# Autodesk Inventor assembly: Light Saber Inventor Native
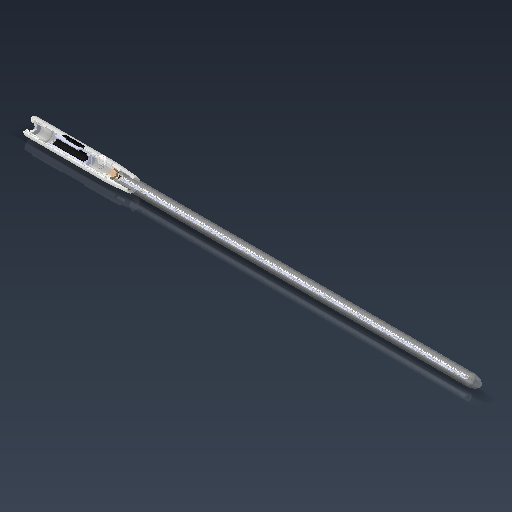
[picture p0: Inventor's stored thumbnail of the model, 512x512]
Saved by Autodesk Inventor 2025.1 (Build 291241000, 241)
## iProperties
Manager: Michael A. Lacey
Company: Personal
Created: 2024-08-20
Part Number: Light Saber Inventor Native
Document SubType Name: Assembly
Designer: Michael A. Lacey
Project: Light Saber
Description: Inventor Recreation
Engineer: Michael A. Lacey
Mass: 701.982 g
Surface Area: 4005.26 cm^2
Volume: 506.243 cm^3
Density: 1.38665 g/cm^3
Author: Michael A. Lacey
Title: LightSaber
Subject: PropBody
## Documents named in this file (12)
- E:\Michael\Documents\GitHub Repos\LightSaber\CAD Files\Rev 3 - Most recent (i think)\Inventor\inventorNative.iam
- E:\Michael\Documents\GitHub Repos\LightSaber\CAD Files\Rev 3 - Most recent (i think)\Inventor\InventorNativeCentralControl.ipt
- E:\Michael\Documents\GitHub Repos\LightSaber\CAD Files\Rev 3 - Most recent (i think)\Inventor\InventorNativeEmitter.ipt
- E:\Michael\Documents\GitHub Repos\LightSaber\CAD Files\Rev 3 - Most recent (i think)\Inventor\InventorNativeNewHilt.ipt
- E:\Michael\Documents\GitHub Repos\LightSaber\CAD Files\Rev 3 - Most recent (i think)\Inventor\PommelPart.ipt
- E:\Michael\Documents\GitHub Repos\LightSaber\CAD Files\Rev 3 - Most recent (i think)\Inventor\PCB HOlder.ipt
- E:\Michael\Documents\GitHub Repos\LightSaber\CAD Files\Rev 3 - Most recent (i think)\Inventor\Speaker.ipt
- E:\Michael\Documents\GitHub Repos\LightSaber\CAD Files\Rev 3 - Most recent (i think)\Inventor\BatteryChargerHolder.ipt
- E:\Michael\Documents\GitHub Repos\LightSaber\CAD Files\Rev 3 - Most recent (i think)\Inventor\Battery.ipt
- E:\Michael\Documents\GitHub Repos\LightSaber\CAD Files\Rev 3 - Most recent (i think)\Inventor\TriHolder.ipt
- E:\Michael\Documents\GitHub Repos\LightSaber\CAD Files\Rev 3 - Most recent (i think)\Inventor\LongBlade.iam
- E:\Michael\Documents\GitHub Repos\LightSaber\CAD Files\Rev 3 - Most recent (i think)\Inventor\Adafruit RGB button.ipt
## Components (11 placed, 11 different names)
1. InventorNativeCentralControl:1 — Mate:1, Mate:3, Mate:4, Mate:5, Mate:24, Mate:25
2. InventorNativeEmitter:1 — Mate:2, Mate:3, Mate:5, Mate:6, Mate:10, Mate:11, Mate:22
3. InventorNativeNewHilt:1 — Mate:1, Mate:2, Mate:4, Mate:6, Mate:7, Mate:8, Mate:9, Mate:18, Mate:19, Mate:20, Mate:21
4. PommelPart:1 — Mate:7, Mate:8, Mate:9, Mate:12, Mate:13
5. PCB HOlder:1 — Mate:10, Mate:11, Mate:23
6. Speaker:1 — Mate:12, Mate:13
7. BatteryChargerHolder:1 — Mate:14, Mate:15
8. Battery:1 — Mate:14, Mate:15
9. TriHolder:1 — Mate:18, Mate:19, Mate:20, Mate:21
10. LongBlade:1 [sub-assembly] — Mate:22, Mate:23
11. Adafruit RGB button:1 — Mate:24, Mate:25
## Relationships (23: Mate 23)
- Mate:1: InventorNativeCentralControl:1 ↔ InventorNativeNewHilt:1
- Mate:2: InventorNativeEmitter:1 ↔ InventorNativeNewHilt:1
- Mate:3: InventorNativeCentralControl:1 ↔ InventorNativeEmitter:1
- Mate:4: InventorNativeCentralControl:1 ↔ InventorNativeNewHilt:1
- Mate:5: InventorNativeCentralControl:1 ↔ InventorNativeEmitter:1
- Mate:6: InventorNativeEmitter:1 ↔ InventorNativeNewHilt:1
- Mate:7: InventorNativeNewHilt:1 ↔ PommelPart:1
- Mate:8: InventorNativeNewHilt:1 ↔ PommelPart:1
- Mate:9: InventorNativeNewHilt:1 ↔ PommelPart:1
- Mate:10: InventorNativeEmitter:1 ↔ PCB HOlder:1
- Mate:11: InventorNativeEmitter:1 ↔ PCB HOlder:1
- Mate:12: PommelPart:1 ↔ Speaker:1
- Mate:13: PommelPart:1 ↔ Speaker:1
- Mate:14: BatteryChargerHolder:1 ↔ Battery:1
- Mate:15 (0.508 mm): BatteryChargerHolder:1 ↔ Battery:1
- Mate:18: InventorNativeNewHilt:1 ↔ TriHolder:1
- Mate:19: InventorNativeNewHilt:1 ↔ TriHolder:1
- Mate:20: InventorNativeNewHilt:1 ↔ TriHolder:1
- Mate:21: InventorNativeNewHilt:1 ↔ TriHolder:1
- Mate:22: InventorNativeEmitter:1 ↔ LongBlade:1
- Mate:23 (1.524 mm): PCB HOlder:1 ↔ LongBlade:1
- Mate:24: InventorNativeCentralControl:1 ↔ Adafruit RGB button:1
- Mate:25: InventorNativeCentralControl:1 ↔ Adafruit RGB button:1
## Named parameters: Finish1_Area = 517.734, Finish2_Area = 517.734, Finish3_Area = 603.294
note: some values were not read from the file. Shown as the stored number, unit unknown: "Finish1_Area", "Finish2_Area", "Finish3_Area".
